# Autodesk Inventor assembly: sk8
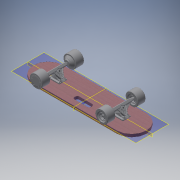
[picture p0: Inventor's stored thumbnail of the model, 180x180]
Saved by Autodesk Inventor 2017 SP1 (Build 210196100, 196)
## iProperties
Part Number: sk8
Material: 一般
Document SubType Name: Assembly
Designer: gisen
Author: gisen
## Documents named in this file (4)
- C:\Users\gisen\Documents\myElectricSk8\CAD\sk8.iam
- C:\Users\gisen\Documents\myElectricSk8\CAD\wheel_kit.iam
- C:\Users\gisen\Documents\myElectricSk8\CAD\board.ipt
- C:\Users\gisen\Documents\myElectricSk8\CAD\wheel_drive_kit.iam
## Components (3 placed, 3 different names)
1. wheel_kit:1 [sub-assembly] — メイト:1, フラッシュ:6
2. board:1 — メイト:1, フラッシュ:6, フラッシュ:7, メイト:3, メイト:4, メイト:5, メイト:6, フラッシュ:8, メイト:7, メイト:8
3. wheel_drive_kit:1 [sub-assembly] — フラッシュ:8, メイト:7, メイト:8
## Relationships (10: Mate 7, Flush 3)
- メイト:1 [Mate]: wheel_kit:1 ↔ board:1
- フラッシュ:6 [Flush]: wheel_kit:1 ↔ board:1
- フラッシュ:7 [Flush]: board:1
- メイト:3 [Mate] (-106 mm): board:1
- メイト:4 [Mate]: board:1
- メイト:5 [Mate]: board:1
- メイト:6 [Mate]: board:1
- フラッシュ:8 [Flush]: board:1 ↔ wheel_drive_kit:1
- メイト:7 [Mate]: board:1 ↔ wheel_drive_kit:1
- メイト:8 [Mate]: board:1 ↔ wheel_drive_kit:1
